# Autodesk Inventor assembly: wh_ass_3_MIR
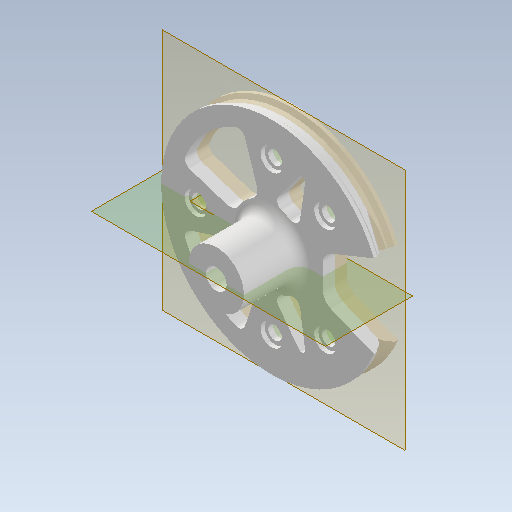
[picture p0: Inventor's stored thumbnail of the model, 512x512]
Saved by Autodesk Inventor 2023 (Build 270158000, 158)
## iProperties
Created: 2021-02-17
Part Number: wh_ass_3_MIR
Document SubType Name: Assembly
Designer: Shuang Peng
Author: Shuang Peng
## Documents named in this file (3)
- D:\projects-3\biped_tiny\hardware\wh_ass_3_MIR.iam
- D:\projects-3\biped_tiny\hardware\screw_holder_2_3_MIR.ipt
- D:\projects-3\biped_tiny\hardware\tendon_wh_3_MIR.ipt
## Components (6 placed, 2 different names)
1. screw_holder_2_3_MIR:1 — Insert:4
2. screw_holder_2_3_MIR:2 — Insert:3
3. screw_holder_2_3_MIR:3 — Insert:5
4. screw_holder_2_3_MIR:4 — Insert:1
5. screw_holder_2_3_MIR:5 — Insert:2
6. tendon_wh_3_MIR:1 — Insert:5, Insert:4, Insert:3, Insert:2, Insert:1
## Relationships (5: Insert 5)
- Insert:5: screw_holder_2_3_MIR:3 ↔ tendon_wh_3_MIR:1
- Insert:4: screw_holder_2_3_MIR:1 ↔ tendon_wh_3_MIR:1
- Insert:3: screw_holder_2_3_MIR:2 ↔ tendon_wh_3_MIR:1
- Insert:2: screw_holder_2_3_MIR:5 ↔ tendon_wh_3_MIR:1
- Insert:1: screw_holder_2_3_MIR:4 ↔ tendon_wh_3_MIR:1
